# Autodesk Inventor assembly: PneumaticWheel_am-0970-2
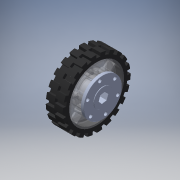
[picture p0: Inventor's stored thumbnail of the model, 180x180]
Saved by Autodesk Inventor 2016 (Build 200138000, 138)
## iProperties
Created: 2011-11-15
Part Number: PneumaticWheel_am-0970-2
Description: STEP AP214
Document SubType Name: Assembly
Designer: gus
Mass: 180.166 g
Surface Area: 846.564 cm^2
Volume: 140.618 cm^3
Density: 1.28124 g/cm^3
Sending System: SolidWorks 2010
Preprocessor: SwSTEP 2.0
Title: Pneumatic Wheel.STEP
Author: Mark
Revision Number: ANY
## Documents named in this file (3)
- \\Mac\Home\Desktop\1510-stronghold-CAD-master\roller wheels\pnumatic wheel\PneumaticWheel_am-0970-2.iam
- \\Mac\Home\Desktop\1510-stronghold-CAD-master\roller wheels\am-0096a+500+Hex+Hub+r2.ipt
- \\Mac\Home\Desktop\1510-stronghold-CAD-master\roller wheels\4-in higrip\4 in HiGrip Wheel.iam
## Components (2 placed, 2 different names)
1. am-0096a+500+Hex+Hub+r2:1 — Mate:1, Mate:2, Mate:3
2. 4 in HiGrip Wheel:1 [sub-assembly] — Mate:1, Mate:2, Mate:3
## Relationships (3: Mate 3)
- Mate:1: am-0096a+500+Hex+Hub+r2:1 ↔ 4 in HiGrip Wheel:1
- Mate:2: am-0096a+500+Hex+Hub+r2:1 ↔ 4 in HiGrip Wheel:1
- Mate:3: am-0096a+500+Hex+Hub+r2:1 ↔ 4 in HiGrip Wheel:1
